# Autodesk Inventor assembly: Spring (McMaster Part #9630K33)
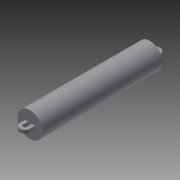
[picture p0: Inventor's stored thumbnail of the model, 180x180]
Saved by Autodesk Inventor 2014 (Build 180170000, 170)
## iProperties
Created: 2014-01-07
Part Number: Spring (McMaster Part #9630K33)
Document SubType Name: Assembly
Designer: Andrew Toennies
Author: Andrew Toennies
## Documents named in this file (2)
- C:\Users\Andrew Toennies\Documents\GitHub\2014buildCAD\Shooter\Spring (McMaster Part #9630K33).iam
- C:\Users\Andrew Toennies\Documents\GitHub\2014buildCAD\Shooter\Spring End.ipt
## Components (2 placed, 1 different names)
1. Spring End:1 — Mate:1, Flush:1, Angle:1, Tangent:1
2. Spring End:2 — Mate:1, Flush:1, Angle:2, Tangent:2
## Relationships (7: Mate 2, Angle 2, Tangent 2, Flush 1)
- Mate:1: Spring End:1 ↔ Spring End:2
- Flush:1: Spring End:1 ↔ Spring End:2
- Angle:1 (0 deg): Spring End:1
- Tangent:1: Spring End:1
- Angle:2 (0 deg): Spring End:2
- Tangent:2: Spring End:2
- Mate:2 (-435.61 mm)
